# Autodesk Inventor assembly: Bulb GU10
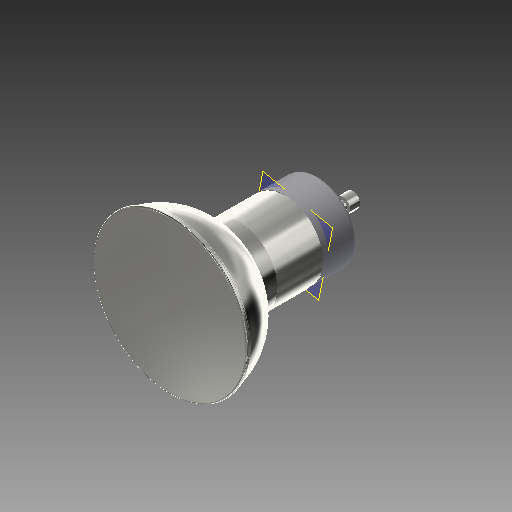
[picture p0: Inventor's stored thumbnail of the model, 512x512]
Saved by Autodesk Inventor 2018.2 (Build 222227000, 227)
## iProperties
Created: 2013-11-23
Part Number: Bulb GU10
Material: Generisch
Description: STEP AP203
Document SubType Name: Assembly
Designer: JochenAlt
Sending System: SolidWorks 2012
Preprocessor: SwSTEP 2.0
Title: GU10_bulb.STEP
Revision Number: ANY
## Documents named in this file (7)
- D:\Projects\concretelamp\CAD\Bulb GU10\Bulb GU10.iam
- D:\Projects\concretelamp\CAD\Bulb GU10\cover_glass.ipt
- D:\Projects\concretelamp\CAD\Bulb GU10\Inlay.ipt
- D:\Projects\concretelamp\CAD\Bulb GU10\Bulb_asm.iam
- D:\Projects\concretelamp\CAD\Bulb GU10\Kontakt-Stück.ipt
- D:\Projects\concretelamp\CAD\Bulb GU10\Klemm-Stück.ipt
- D:\Projects\concretelamp\CAD\LampAddOn.ipt
## Components (6 placed, 6 different names)
1. cover_glass_1 — Fluchtend:1, Fluchtend:2
2. Inlay_2
3. Bulb_asm:1 [sub-assembly]
4. Kontakt-Stück_4 — Fluchtend:3, Passend:1, Passend:2
5. Klemm-Stück_5
6. LampAddOn:1 — Fluchtend:1, Fluchtend:2, Fluchtend:3, Passend:1, Passend:2
## Relationships (5: Flush 3, Mate 2)
- Fluchtend:1 [Flush]: cover_glass_1 ↔ LampAddOn:1
- Fluchtend:2 [Flush]: cover_glass_1 ↔ LampAddOn:1
- Fluchtend:3 [Flush]: Kontakt-Stück_4 ↔ LampAddOn:1
- Passend:1 [Mate] (5 mm): Kontakt-Stück_4 ↔ LampAddOn:1
- Passend:2 [Mate] (5 mm): Kontakt-Stück_4 ↔ LampAddOn:1
